# Autodesk Inventor assembly: 3D_Drucker_v02
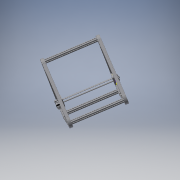
[picture p0: Inventor's stored thumbnail of the model, 180x180]
Saved by Autodesk Inventor 2019 (Build 230136000, 136)
## iProperties
Created: 2018-08-19
Part Number: 3D_Drucker_v02
Document SubType Name: Assembly
Designer: Julia
Author: Julia
## Documents named in this file (5)
- C:\Users\Julia\Documents\Inventor\3d_Drucker_v02\3D_Drucker_v02.iam
- C:\Users\Julia\Documents\Inventor\3d_Drucker_v02\Rahmen.iam
- C:\Users\Julia\Documents\Inventor\3d_Drucker_v02\Y_Führung.iam
- C:\Users\Julia\Documents\Inventor\3d_Drucker_v02\X_Führung.iam
- C:\Users\Julia\Documents\Inventor\3d_Drucker_v02\Schrittmotor_Nema_17.ipt
## Components (6 placed, 4 different names)
1. Rahmen:1 [sub-assembly] — Mate:1, Mate:2, Mate:3, Mate:4, Mate:5, Mate:6, Mate:7, Mate:8, Mate:11, Mate:12, Mate:13, Mate:14, Mate:15, Mate:16
2. Y_Führung:1 [sub-assembly] — Mate:1, Mate:2, Mate:3, Mate:4, Mate:10
3. Y_Führung:2 [sub-assembly] — Mate:5, Mate:6, Mate:7, Mate:8, Mate:9
4. X_Führung:1 [sub-assembly] — Mate:9, Mate:10
5. Schrittmotor_Nema_17:1 — Mate:11, Mate:12, Mate:13
6. Schrittmotor_Nema_17:2 — Mate:14, Mate:15, Mate:16
## Relationships (16: Mate 16)
- Mate:1: Rahmen:1 ↔ Y_Führung:1
- Mate:2: Rahmen:1 ↔ Y_Führung:1
- Mate:3: Rahmen:1 ↔ Y_Führung:1
- Mate:4: Rahmen:1 ↔ Y_Führung:1
- Mate:5: Rahmen:1 ↔ Y_Führung:2
- Mate:6: Rahmen:1 ↔ Y_Führung:2
- Mate:7: Rahmen:1 ↔ Y_Führung:2
- Mate:8: Rahmen:1 ↔ Y_Führung:2
- Mate:9: Y_Führung:2 ↔ X_Führung:1
- Mate:10: Y_Führung:1 ↔ X_Führung:1
- Mate:11: Rahmen:1 ↔ Schrittmotor_Nema_17:1
- Mate:12: Rahmen:1 ↔ Schrittmotor_Nema_17:1
- Mate:13: Rahmen:1 ↔ Schrittmotor_Nema_17:1
- Mate:14: Rahmen:1 ↔ Schrittmotor_Nema_17:2
- Mate:15: Rahmen:1 ↔ Schrittmotor_Nema_17:2
- Mate:16: Rahmen:1 ↔ Schrittmotor_Nema_17:2
